# Autodesk Inventor assembly: teljes3
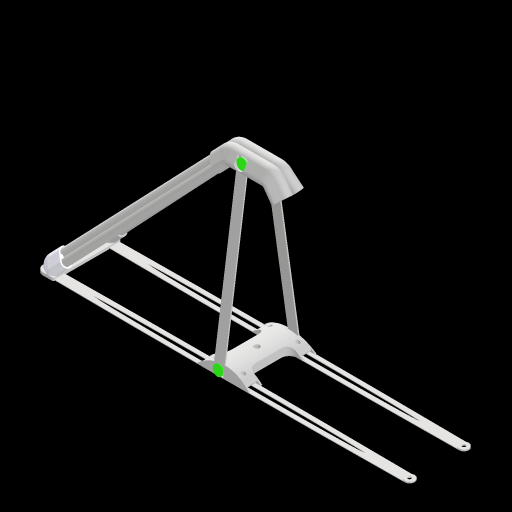
[picture p0: Inventor's stored thumbnail of the model, 512x512]
Saved by Autodesk Inventor 2023 (Build 270158000, 158)
## iProperties
Created: 2022-11-11
Part Number: teljes3
Document SubType Name: Assembly
Designer: gd1
Author: gd1
## Documents named in this file (9)
- C:\Users\gd1\3D Objects\3D nagyteherbírású híd\Híd\H-d\teljes6.iam
- C:\Users\gd1\3D Objects\3D nagyteherbírású híd\Híd\H-d\45 fok középre_talp.ipt
- C:\Users\gd1\3D Objects\3D nagyteherbírású híd\Híd\H-d\palca 325mm.ipt
- C:\Users\gd1\3D Objects\3D nagyteherbírású híd\Híd\H-d\45 fok kozepcsati.ipt.iam
- C:\Users\gd1\3D Objects\3D nagyteherbírású híd\Híd\H-d\közepső szalag 1.ipt
- C:\Users\gd1\3D Objects\3D nagyteherbírású híd\Híd\H-d\kozepso_csomopont.ipt
- C:\Users\gd1\3D Objects\3D nagyteherbírású híd\Híd\H-d\tipli.ipt
- C:\Users\gd1\3D Objects\3D nagyteherbírású híd\Híd\H-d\szalag3.ipt
- 45 fok kozepcsati.ipt
## Components (15 placed, 7 different names)
1. 45 fok középre_talp:1 — Rotational:1, Rotational:2, Rotational:19, Rotational:20
2. palca 325mm:1 — Rotational:2
3. palca 325mm:2 — Rotational:1
4. 45 fok kozepcsati.ipt:1 [sub-assembly] — Rotational:10, Rotational:16
5. közepső szalag 1:2 — Rotational:10, Rotational:14, Rotational:15
6. kozepso_csomopont:1
7. tipli:2 — Rotational:18
8. tipli:3 — Rotational:15
9. tipli:5
10. tipli:6
11. tipli:7 — Rotational:17
12. tipli:8 — Rotational:14
13. közepső szalag 1:3 — Rotational:16, Rotational:17, Rotational:18
14. szalag3:1 — Rotational:19
15. szalag3:2 — Rotational:20
## Relationships (10: RevoluteJoint 10)
- Rotational:1 [RevoluteJoint]: 45 fok középre_talp:1 ↔ palca 325mm:2
- Rotational:2 [RevoluteJoint]: 45 fok középre_talp:1 ↔ palca 325mm:1
- Rotational:10 [RevoluteJoint]: 45 fok kozepcsati.ipt:1 ↔ közepső szalag 1:2
- Rotational:14 [RevoluteJoint]: közepső szalag 1:2 ↔ tipli:8
- Rotational:15 [RevoluteJoint]: közepső szalag 1:2 ↔ tipli:3
- Rotational:16 [RevoluteJoint]: 45 fok kozepcsati.ipt:1 ↔ közepső szalag 1:3
- Rotational:17 [RevoluteJoint]: tipli:7 ↔ közepső szalag 1:3
- Rotational:18 [RevoluteJoint]: tipli:2 ↔ közepső szalag 1:3
- Rotational:19 [RevoluteJoint]: 45 fok középre_talp:1 ↔ szalag3:1
- Rotational:20 [RevoluteJoint]: 45 fok középre_talp:1 ↔ szalag3:2
